# Autodesk Inventor assembly: YaxisAssem
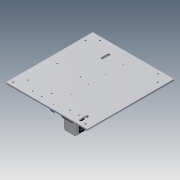
[picture p0: Inventor's stored thumbnail of the model, 180x180]
Saved by Autodesk Inventor 2014 (Build 180170000, 170)
## iProperties
Created: 2015-02-16
Part Number: YaxisAssem
Document SubType Name: Assembly
Designer: Peele
Author: Peele
## Documents named in this file (5)
- E:\Copy\DLP\PandaPrint\CustomParts\YaxisAssem.iam
- E:\Copy\DLP\PandaPrint\CustomParts\NewBackPlate.ipt
- E:\Copy\DLP\PandaPrint\StockParts\Rail.ipt
- E:\Copy\DLP\PandaPrint\StockParts\Rail\Rail-02.ipt
- E:\Copy\DLP\PandaPrint\SubAssem\StepperWithMount-210mm.iam
## Components (3 placed, 3 different names)
1. NewBackPlate:1 — Mate:1, Mate:2, Flush:1, Mate:3, Flush:5, Mate:5, Mate:6, Flush:6, Tangent:1
2. Rail-02:1 — Mate:3, Flush:5, Mate:5
3. StepperWithMount-210mm:1 [sub-assembly] — Mate:6, Flush:6, Tangent:1
## Relationships (9: Mate 5, Flush 3, Tangent 1)
- Mate:1: NewBackPlate:1
- Mate:2: NewBackPlate:1
- Flush:1: NewBackPlate:1
- Mate:3: NewBackPlate:1 ↔ Rail-02:1
- Flush:5 (-40 mm): NewBackPlate:1 ↔ Rail-02:1
- Mate:5: NewBackPlate:1 ↔ Rail-02:1
- Mate:6: NewBackPlate:1 ↔ StepperWithMount-210mm:1
- Flush:6: NewBackPlate:1 ↔ StepperWithMount-210mm:1
- Tangent:1: NewBackPlate:1 ↔ StepperWithMount-210mm:1
